# Autodesk Inventor assembly: yield_assemble
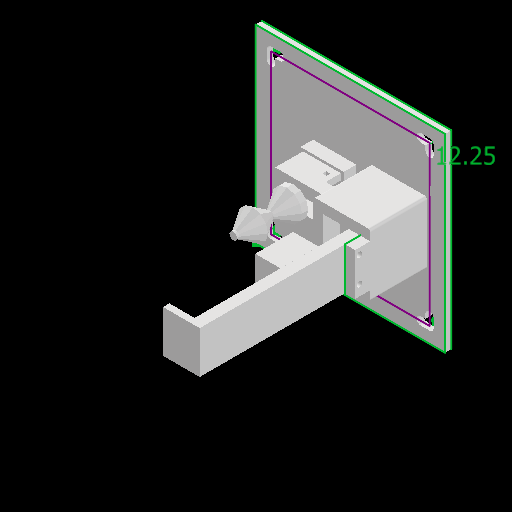
[picture p0: Inventor's stored thumbnail of the model, 512x512]
Saved by Autodesk Inventor 2025.1 (Build 291241000, 241)
## iProperties
Created: 2024-08-22
Part Number: yield_assemble
Document SubType Name: Assembly
Designer: ojs08
Author: ojs08
## Documents named in this file (6)
- C:\Users\ojs08\OneDrive\바탕 화면\SKKU\3학년 1학기\여름방학 URP\yield_assemble.iam
- C:\Users\ojs08\OneDrive\바탕 화면\SKKU\3학년 1학기\여름방학 URP\yield_bed.ipt
- C:\Users\ojs08\OneDrive\바탕 화면\SKKU\3학년 1학기\여름방학 URP\linear_actuator.ipt
- C:\Users\ojs08\OneDrive\바탕 화면\SKKU\3학년 1학기\여름방학 URP\linear_motor.ipt
- C:\Users\ojs08\OneDrive\문서\카카오톡 받은 파일\valve_mount.ipt
- C:\Users\ojs08\OneDrive\문서\카카오톡 받은 파일\finger.ipt
## Components (5 placed, 5 different names)
1. valve_mount:1 — 메이트:8, 메이트:9, 메이트:10, 메이트:11
2. yield_bed:1 — 메이트:8, 메이트:9, 메이트:10, 메이트:12, 메이트:13, 메이트:14
3. finger:1 — 메이트:11
4. linear_actuator:1 — 메이트:15, 메이트:16
5. linear_motor:1 — 메이트:12, 메이트:13, 메이트:14, 메이트:15, 메이트:16
## Relationships (9: Mate 9)
- 메이트:8 [Mate]: valve_mount:1 ↔ yield_bed:1
- 메이트:9 [Mate]: valve_mount:1 ↔ yield_bed:1
- 메이트:10 [Mate]: valve_mount:1 ↔ yield_bed:1
- 메이트:11 [Mate]: valve_mount:1 ↔ finger:1
- 메이트:12 [Mate]: yield_bed:1 ↔ linear_motor:1
- 메이트:13 [Mate]: yield_bed:1 ↔ linear_motor:1
- 메이트:14 [Mate]: yield_bed:1 ↔ linear_motor:1
- 메이트:15 [Mate]: linear_actuator:1 ↔ linear_motor:1
- 메이트:16 [Mate]: linear_actuator:1 ↔ linear_motor:1
